# Autodesk Inventor assembly: CAR_015_CarouselTensionerAssembly
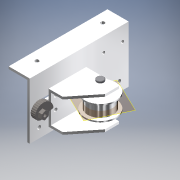
[picture p0: Inventor's stored thumbnail of the model, 180x180]
Saved by Autodesk Inventor 2018 (Build 220112000, 112)
## iProperties
Created: 2020-02-01
Part Number: CAR_015_CarouselTensionerAssembly
Document SubType Name: Assembly
Designer: user
Author: user
## Documents named in this file (7)
- C:\Users\user\Documents\GrabCAD\New folder\Build season\CAR_015_CarouselTensionerAssembly.iam
- C:\Users\user\Documents\GrabCAD\New folder\Build season\CAR_014_CarouselTensionerPulley.ipt
- C:\Users\user\Documents\GrabCAD\New folder\Build season\CAR_016_TensionerMount.ipt
- C:\Users\user\Documents\GrabCAD\New folder\Build season\CAR_017_57155K305_STAINLESS STEEL BALL BEARING.ipt
- C:\Users\user\Documents\GrabCAD\New folder\Build season\CAR_018_98306A167_STEEL CLEVIS PIN.ipt
- C:\Users\user\Documents\GrabCAD\New folder\Build season\CAR_019_TensionerLBracket.ipt
- C:\Users\user\Documents\GrabCAD\New folder\Build season\CAR_020_217-3431_(CAM).ipt
## Components (7 placed, 6 different names)
1. CAR_014_CarouselTensionerPulley:1 — Insert:1, Insert:2, Mate:3
2. CAR_016_TensionerMount:1 — Insert:3, Mate:2, Flush:1, Mate:3
3. CAR_017_57155K305_STAINLESS STEEL BALL BEARING:1 — Insert:1, Mate:1
4. CAR_017_57155K305_STAINLESS STEEL BALL BEARING:2 — Insert:2
5. CAR_018_98306A167_STEEL CLEVIS PIN:1 — Insert:3, Mate:1
6. CAR_019_TensionerLBracket:1 — Mate:2, Flush:1, Insert:4
7. CAR_020_217-3431_(CAM):1 — Insert:4
## Relationships (8: Insert 4, Mate 3, Flush 1)
- Insert:1: CAR_014_CarouselTensionerPulley:1 ↔ CAR_017_57155K305_STAINLESS STEEL BALL BEARING:1
- Insert:2: CAR_014_CarouselTensionerPulley:1 ↔ CAR_017_57155K305_STAINLESS STEEL BALL BEARING:2
- Insert:3: CAR_016_TensionerMount:1 ↔ CAR_018_98306A167_STEEL CLEVIS PIN:1
- Mate:1: CAR_017_57155K305_STAINLESS STEEL BALL BEARING:1 ↔ CAR_018_98306A167_STEEL CLEVIS PIN:1
- Mate:2: CAR_016_TensionerMount:1 ↔ CAR_019_TensionerLBracket:1
- Flush:1 (24.4094 mm): CAR_016_TensionerMount:1 ↔ CAR_019_TensionerLBracket:1
- Mate:3 (9.525 mm): CAR_014_CarouselTensionerPulley:1 ↔ CAR_016_TensionerMount:1
- Insert:4: CAR_019_TensionerLBracket:1 ↔ CAR_020_217-3431_(CAM):1
